# Autodesk Inventor assembly: WPS
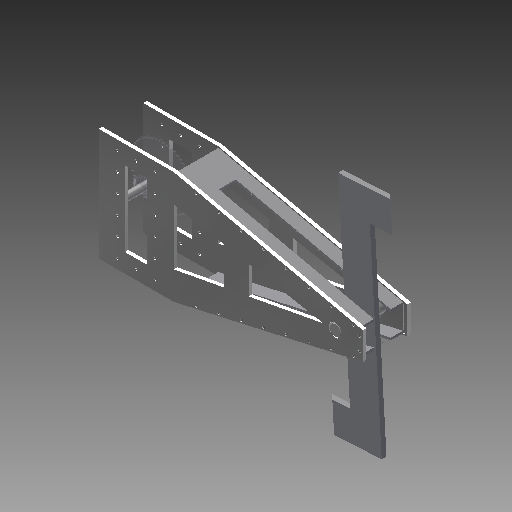
[picture p0: Inventor's stored thumbnail of the model, 512x512]
Saved by Autodesk Inventor 2017 (Build 210142000, 142)
## iProperties
Created: 2016-12-06
Part Number: WPS
Document SubType Name: Assembly
Designer: aesen
Author: aesen
## Documents named in this file (4)
- C:\Users\aesen\Design\newassembly\WPS.iam
- C:\Users\aesen\Design\newassembly\W1sup.ipt
- C:\Users\aesen\Design\newassembly\sidesupport.ipt
- C:\Users\aesen\Design\newassembly\W1chain\Assembly6.iam
## Components (5 placed, 3 different names)
1. W1sup:1 — Mate:1, Mate:2, Mate:3, Mate:4, Mate:5, Mate:6, Insert:1
2. sidesupport:1 — Mate:1, Mate:2, Mate:3
3. sidesupport:2 — Mate:4, Mate:5, Mate:6, Mate:7, Mate:8
4. Assembly6:1 [sub-assembly] — Insert:1
5. W1sup:2 — Mate:7, Mate:8
## Relationships (9: Mate 8, Insert 1)
- Mate:1: W1sup:1 ↔ sidesupport:1
- Mate:2: W1sup:1 ↔ sidesupport:1
- Mate:3: W1sup:1 ↔ sidesupport:1
- Mate:4: W1sup:1 ↔ sidesupport:2
- Mate:5: W1sup:1 ↔ sidesupport:2
- Mate:6: W1sup:1 ↔ sidesupport:2
- Insert:1 (-10.16 mm): W1sup:1 ↔ Assembly6:1
- Mate:7: sidesupport:2 ↔ W1sup:2
- Mate:8: sidesupport:2 ↔ W1sup:2
